# Autodesk Inventor assembly: Assembly
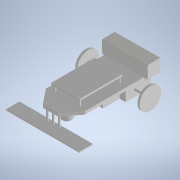
[picture p0: Inventor's stored thumbnail of the model, 180x180]
Saved by Autodesk Inventor 2022 (Build 260153000, 153)
## iProperties
Created: 2021-07-05
Part Number: Assembly
Document SubType Name: Assembly
Designer: ken
Author: ken
## Documents named in this file (10)
- G:\マイドライブ\Projects\lineTracer\inventor\Assembly.iam
- G:\マイドライブ\Projects\lineTracer\inventor\double_gearbox.ipt
- G:\マイドライブ\Projects\lineTracer\inventor\tire.ipt
- G:\マイドライブ\Projects\lineTracer\inventor\ballcaster.ipt
- G:\マイドライブ\Projects\lineTracer\inventor\sensorPCB.ipt
- G:\マイドライブ\Projects\lineTracer\inventor\mainBoard.ipt
- G:\マイドライブ\Projects\lineTracer\inventor\spacer-10mm.ipt
- G:\マイドライブ\Projects\lineTracer\inventor\spacer-20mm.ipt
- G:\マイドライブ\Projects\lineTracer\inventor\batteryBox.ipt
- G:\マイドライブ\Projects\lineTracer\inventor\body.ipt
## Components (15 placed, 9 different names)
1. tire:1 — 挿入:2
2. tire:2 — 挿入:1
3. double_gearbox:1 — 挿入:1, 挿入:2, 挿入:30
4. ballcaster:1 — 挿入:24, 挿入:25
5. sensorPCB:1 — 挿入:19, 挿入:20, 挿入:21
6. mainBoard:1 — 挿入:12, 挿入:13, 挿入:14, 挿入:15
7. spacer-10mm:1 — 挿入:12, 挿入:29
8. spacer-10mm:2 — 挿入:13
9. spacer-10mm:3 — 挿入:15
10. spacer-10mm:4 — 挿入:14, 挿入:28
11. spacer-20mm:1 — 挿入:21, 挿入:23
12. spacer-20mm:2 — 挿入:20
13. spacer-20mm:3 — 挿入:19, 挿入:22
14. batteryBox:1
15. body:1 — 挿入:22, 挿入:23, 挿入:24, 挿入:25, 挿入:28, 挿入:29, 挿入:30
## Relationships (16: Insert 16)
- 挿入:1 [Insert]: tire:2 ↔ double_gearbox:1
- 挿入:2 [Insert]: tire:1 ↔ double_gearbox:1
- 挿入:12 [Insert]: mainBoard:1 ↔ spacer-10mm:1
- 挿入:13 [Insert]: mainBoard:1 ↔ spacer-10mm:2
- 挿入:14 [Insert]: mainBoard:1 ↔ spacer-10mm:4
- 挿入:15 [Insert]: mainBoard:1 ↔ spacer-10mm:3
- 挿入:19 [Insert]: sensorPCB:1 ↔ spacer-20mm:3
- 挿入:20 [Insert]: sensorPCB:1 ↔ spacer-20mm:2
- 挿入:21 [Insert]: sensorPCB:1 ↔ spacer-20mm:1
- 挿入:22 [Insert]: spacer-20mm:3 ↔ body:1
- 挿入:23 [Insert]: spacer-20mm:1 ↔ body:1
- 挿入:24 [Insert]: ballcaster:1 ↔ body:1
- 挿入:25 [Insert]: ballcaster:1 ↔ body:1
- 挿入:28 [Insert]: spacer-10mm:4 ↔ body:1
- 挿入:29 [Insert]: spacer-10mm:1 ↔ body:1
- 挿入:30 [Insert]: double_gearbox:1 ↔ body:1
